# Autodesk Inventor assembly: big pulley
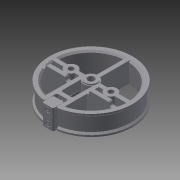
[picture p0: Inventor's stored thumbnail of the model, 180x180]
Saved by Autodesk Inventor 2014 (Build 180170000, 170)
## iProperties
Created: 2013-10-14
Part Number: big pulley
Document SubType Name: Assembly
Designer: employee
Author: employee
## Documents named in this file (6)
- \\GRISTLE\speco\GitHub\ConceptFORGE\Wally\big pulley.iam
- \\GRISTLE\speco\GitHub\ConceptFORGE\Wally\big pulley.ipt
- \\GRISTLE\speco\GitHub\ConceptFORGE\Wally\m3 nut.ipt
- \\GRISTLE\speco\GitHub\ConceptFORGE\Wally\string tensioner.ipt
- \\GRISTLE\speco\GitHub\ConceptFORGE\Wally\M3x35.ipt
- \\GRISTLE\speco\GitHub\ConceptFORGE\Wally\washer.ipt
## Components (7 placed, 5 different names)
1. big pulley:1 — Insert:1, Insert:2, Angle:1, Angle:2, Insert:3, Mate:1, Insert:6
2. Hex Nut Metric M3 x 0.5:1 — Insert:2, Angle:2
3. Hex Nut Metric M3 x 0.5:2 — Insert:1, Angle:1
4. string tensioner:1 — Insert:3, Mate:1, Insert:4, Insert:5
5. M3x35:1 — Insert:5
6. M3x35:2 — Insert:4
7. washer:1 — Insert:6
## Relationships (9: Insert 6, Angle 2, Mate 1)
- Insert:1: big pulley:1 ↔ Hex Nut Metric M3 x 0.5:2
- Insert:2: big pulley:1 ↔ Hex Nut Metric M3 x 0.5:1
- Angle:1 (0 deg): big pulley:1 ↔ Hex Nut Metric M3 x 0.5:2
- Angle:2 (0 deg): big pulley:1 ↔ Hex Nut Metric M3 x 0.5:1
- Insert:3 (5 mm): big pulley:1 ↔ string tensioner:1
- Mate:1: big pulley:1 ↔ string tensioner:1
- Insert:4: string tensioner:1 ↔ M3x35:2
- Insert:5: string tensioner:1 ↔ M3x35:1
- Insert:6: big pulley:1 ↔ washer:1
